# Autodesk Inventor assembly: PIHTI-for-Boron
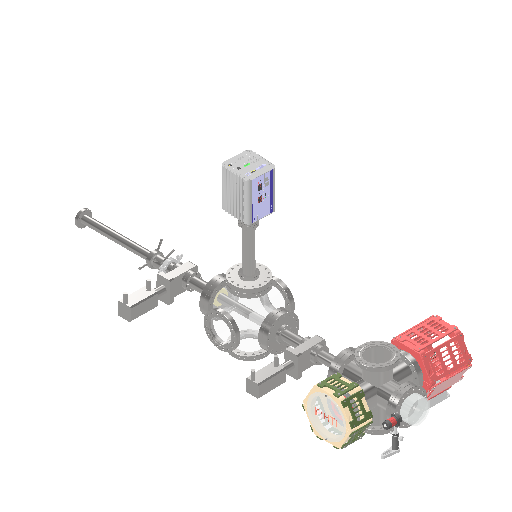
[picture p0: Inventor's stored thumbnail of the model, 512x512]
Saved by Autodesk Inventor 2026.2 (Build 302298000, 298)
## iProperties
Created: 2024-05-09
Part Number: PIHTI-for-Boron
Document SubType Name: Assembly
Designer: kuzmin
Mass: 19614.5 g
Surface Area: 13609.5 cm^2
Volume: 3689.47 cm^3
Density: 5.31636 g/cm^3
Author: kuzmin
## Documents named in this file (25)
- D:\repos\PIHTI\Plasma Vessel\PIHTI-for-Boron.iam
- D:\repos\PIHTI\Plasma Vessel\Plasma-vacuum-cross\Plasma-vacuum-vessel-152IC-cross.iam
- D:\repos\PIHTI\Plasma Vessel\Plasma-Flange-2024\cathode-box-on-a-flange.iam
- D:\repos\PIHTI\Plasma Vessel\Cathode-Flange-Cage\CathodeCage.iam
- D:\repos\PIHTI\Plasma Vessel\Cathode-Anode-Flange\Cathode-Anode-70IC-flange-with-feeds.iam
- D:\repos\PIHTI\Plasma Vessel\Plasma-Box\Plasma-box-hayashi-aka-upgrade.iam
- D:\repos\PIHTI\ContentCenter\Fastners\M3x8-SHCS.ipt
- D:\repos\PIHTI\Plasma Vessel\Plasma-Box\probe-gate-with-spindel.iam
- D:\repos\PIHTI\Plasma Vessel\Cathode-Anode-Flange\cf70_spacer.ipt
- D:\repos\PIHTI\Plasma Vessel\Plasma-Box\anode-on-flange.iam
- D:\repos\PIHTI\Plasma Vessel\entrance-mesh-assembly.iam
- D:\repos\PIHTI\Plasma Vessel\Oring-probe-flange-with-GV.iam
- D:\repos\PIHTI\Plasma Vessel\Plasma-Box-Support.ipt
- D:\repos\PIHTI\Plasma Vessel\probe-port-mesh-welded.iam
- D:\repos\PIHTI\Plasma Vessel\Mesh-mounting-help.ipt
- D:\repos\PIHTI\Plasma Vessel\Cathode-Flange-Cage\Short-Cage.iam
- D:\repos\PIHTI\ContentCenter\CF-parts\CF-Flanges\CF_152-70.ipt
- D:\repos\PIHTI\ContentCenter\CF-parts\CF70-nipple\CF70-nipple.iam
- D:\repos\PIHTI\ContentCenter\CF-parts\CF70-gate-valve\Gatevalve_70_pneumatic.iam
- D:\repos\PIHTI\BoronProbe\BoronProbe.iam
- D:\repos\PIHTI\ContentCenter\ulvac\Qulee_BGM2-102_202.ipt
- D:\repos\PIHTI\Plasma Vessel\Plasma-vacuum-cross\UFC-152.ipt
- C:\Users\queez\Dropbox\Drawings\PIHTI\Plasma Vessel\Plasma-vacuum-cross\UFC.ipt
- D:\repos\PIHTI\BoronProbe\GlassPort-idea.ipt
- D:\repos\PIHTI\ContentCenter\Optics\collimator.iam
## Components (34 placed, 23 different names)
1. Plasma-vacuum-vessel-152IC-cross:1 [sub-assembly] — メイト:1, フラッシュ:1, フラッシュ:2, 回転:1, メイト:15, メイト:16, リジッド:17, リジッド:18, メイト:21, 回転:21, フラッシュ:4
2. cathode-box-on-a-flange:1 [sub-assembly] — 回転:1, 回転:2, メイト:2, メイト:5, リジッド:10
3. CathodeCage:1 [sub-assembly] — 回転:2
4. Cathode-Anode-70IC-flange-with-feeds:1 [sub-assembly] — メイト:2, メイト:5, メイト:6
5. Plasma-box-hayashi-aka-upgrade:1 [sub-assembly] — メイト:3, メイト:4, Hinge Angle, メイト:7, メイト:8, メイト:9, メイト:13, メイト:17
6. probe-gate-with-spindel:1 [sub-assembly] — メイト:3, メイト:4, Hinge Angle
7. cf70_spacer:1 — リジッド:10, メイト:6
8. anode-on-flange:1 [sub-assembly] — メイト:7, メイト:8, メイト:9, リジッド:11, リジッド:12, リジッド:13, リジッド:14
9. entrance-mesh-assembly:1 [sub-assembly] — メイト:13, メイト:17, メイト:19
10. Oring-probe-flange-with-GV:1 [sub-assembly] — メイト:15, リジッド:16, 回転:3
11. Plasma-Box-Support:1 — メイト:16, フラッシュ:3
12. probe-port-mesh-welded:1 [sub-assembly] — メイト:19
13. Mesh-mounting-help:1 — リジッド:16
14. Short-Cage:1 [sub-assembly] — リジッド:17
15. Plasma-vacuum-vessel-152IC-cross:2 [sub-assembly] — 回転:20, 回転:3, リジッド:25
16. CF_152-70:1 — リジッド:18, メイト:20, リジッド:21
17. CF_152-70:2 — 回転:20, メイト:20, リジッド:24
18. CF70-nipple:1 [sub-assembly] — リジッド:21, リジッド:22
19. CF70-nipple:2 [sub-assembly] — リジッド:23, リジッド:24
20. Gatevalve_70_pneumatic:1 [sub-assembly] — リジッド:22, リジッド:23
21. BoronProbe:1 [sub-assembly] — メイト:21
22. CF_152-70:3 — リジッド:25, 回転:4
23. Qulee_BGM2-102_202:1 — 回転:4
24. UFC-152:1 — 回転:21, リジッド:26
25. GlassPort-idea:1 — リジッド:26
26. collimator:1 [sub-assembly] — フラッシュ:4
27. SS ISO 4762 M3 x 8:5 — リジッド:11
28. SS ISO 4762 M3 x 8:6 — リジッド:12
29. SS ISO 4762 M3 x 8:7 — リジッド:14
30. SS ISO 4762 M3 x 8:8 — リジッド:13
31. SS ISO 4762 M3 x 8:1
32. SS ISO 4762 M3 x 8:2
33. SS ISO 4762 M3 x 8:3
34. SS ISO 4762 M3 x 8:4
## Relationships (42: Mate 17, WeldJoint 14, RevoluteJoint 6, Flush 4, Angle 1)
- メイト:1 [Mate]: Plasma-vacuum-vessel-152IC-cross:1
- フラッシュ:1 [Flush]: Plasma-vacuum-vessel-152IC-cross:1
- フラッシュ:2 [Flush]: Plasma-vacuum-vessel-152IC-cross:1
- 回転:1 [RevoluteJoint]: Plasma-vacuum-vessel-152IC-cross:1 ↔ cathode-box-on-a-flange:1
- 回転:2 [RevoluteJoint]: cathode-box-on-a-flange:1 ↔ CathodeCage:1
- メイト:2 [Mate]: cathode-box-on-a-flange:1 ↔ Cathode-Anode-70IC-flange-with-feeds:1
- メイト:3 [Mate]: Plasma-box-hayashi-aka-upgrade:1 ↔ probe-gate-with-spindel:1
- メイト:4 [Mate]: Plasma-box-hayashi-aka-upgrade:1 ↔ probe-gate-with-spindel:1
- Hinge Angle [Angle] (45 deg): Plasma-box-hayashi-aka-upgrade:1 ↔ probe-gate-with-spindel:1
- メイト:5 [Mate]: cathode-box-on-a-flange:1 ↔ Cathode-Anode-70IC-flange-with-feeds:1
- リジッド:10 [WeldJoint]: cathode-box-on-a-flange:1 ↔ cf70_spacer:1
- メイト:6 [Mate]: Cathode-Anode-70IC-flange-with-feeds:1 ↔ cf70_spacer:1
- メイト:7 [Mate]: Plasma-box-hayashi-aka-upgrade:1 ↔ anode-on-flange:1
- メイト:8 [Mate]: Plasma-box-hayashi-aka-upgrade:1 ↔ anode-on-flange:1
- メイト:9 [Mate]: Plasma-box-hayashi-aka-upgrade:1 ↔ anode-on-flange:1
- リジッド:11 [WeldJoint]: anode-on-flange:1 ↔ SS ISO 4762 M3 x 8:5
- リジッド:12 [WeldJoint]: anode-on-flange:1 ↔ SS ISO 4762 M3 x 8:6
- リジッド:13 [WeldJoint]: anode-on-flange:1 ↔ SS ISO 4762 M3 x 8:8
- リジッド:14 [WeldJoint]: anode-on-flange:1 ↔ SS ISO 4762 M3 x 8:7
- [Mate]: Plasma-vacuum-vessel-152IC-cross:1 ↔ Oring-probe-flange-with-GV:1
- メイト:13 [Mate]: Plasma-box-hayashi-aka-upgrade:1 ↔ entrance-mesh-assembly:1
- メイト:15 [Mate]: Plasma-vacuum-vessel-152IC-cross:1 ↔ Oring-probe-flange-with-GV:1
- メイト:16 [Mate]: Plasma-vacuum-vessel-152IC-cross:1 ↔ Plasma-Box-Support:1
- フラッシュ:3 [Flush]: Plasma-Box-Support:1
- メイト:17 [Mate]: Plasma-box-hayashi-aka-upgrade:1 ↔ entrance-mesh-assembly:1
- リジッド:16 [WeldJoint]: Oring-probe-flange-with-GV:1 ↔ Mesh-mounting-help:1
- リジッド:17 [WeldJoint]: Plasma-vacuum-vessel-152IC-cross:1 ↔ Short-Cage:1
- メイト:19 [Mate]: entrance-mesh-assembly:1 ↔ probe-port-mesh-welded:1
- リジッド:18 [WeldJoint]: Plasma-vacuum-vessel-152IC-cross:1 ↔ CF_152-70:1
- 回転:20 [RevoluteJoint]: Plasma-vacuum-vessel-152IC-cross:2 ↔ CF_152-70:2
- メイト:20 [Mate]: CF_152-70:1 ↔ CF_152-70:2
- 回転:3 [RevoluteJoint]: Oring-probe-flange-with-GV:1 ↔ Plasma-vacuum-vessel-152IC-cross:2
- リジッド:21 [WeldJoint]: CF_152-70:1 ↔ CF70-nipple:1
- リジッド:22 [WeldJoint]: CF70-nipple:1 ↔ Gatevalve_70_pneumatic:1
- リジッド:23 [WeldJoint]: CF70-nipple:2 ↔ Gatevalve_70_pneumatic:1
- リジッド:24 [WeldJoint]: CF_152-70:2 ↔ CF70-nipple:2
- メイト:21 [Mate]: Plasma-vacuum-vessel-152IC-cross:1 ↔ BoronProbe:1
- リジッド:25 [WeldJoint]: Plasma-vacuum-vessel-152IC-cross:2 ↔ CF_152-70:3
- 回転:4 [RevoluteJoint]: CF_152-70:3 ↔ Qulee_BGM2-102_202:1
- 回転:21 [RevoluteJoint]: Plasma-vacuum-vessel-152IC-cross:1 ↔ UFC-152:1
- リジッド:26 [WeldJoint]: UFC-152:1 ↔ GlassPort-idea:1
- フラッシュ:4 [Flush] (20 mm): Plasma-vacuum-vessel-152IC-cross:1 ↔ collimator:1
